# Autodesk Inventor assembly: ASY PNS 1780 FDS 1200x90 Top elbow
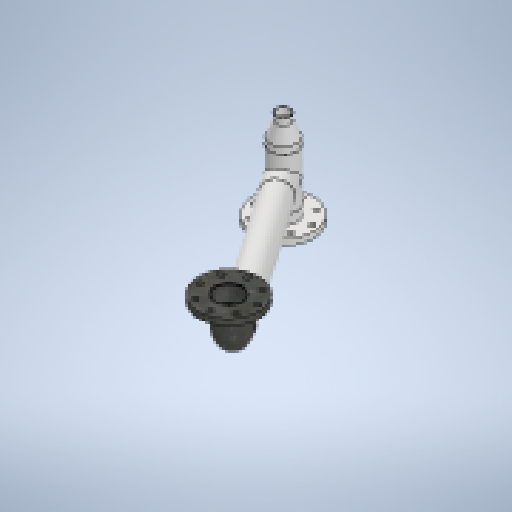
[picture p0: Inventor's stored thumbnail of the model, 512x512]
Saved by Autodesk Inventor 2025.1 (Build 291241020, 241B)
## iProperties
Created: 2025-07-10
Part Number: ASY PNS 1780 FDS 1200x90 Top elbow
Document SubType Name: Assembly
Designer: user
Author: user
## Documents named in this file (7)
- C:\Users\user\YandexDisk-badmisterfox\home pc\Inventor\PNS2-Panaevsk\Filter D1200\ASY PNS 1780 FDS 1200x90 Top elbow.iam
- C:\Users\user\YandexDisk-badmisterfox\home pc\Inventor\PNS2-Panaevsk\Filter D1000\DIN 2576 Slip-On Flange for Welding Series 1 (ISO) - PN 10 80 x 88.9.ipt
- C:\Users\user\YandexDisk-badmisterfox\home pc\Inventor\PNS2-Panaevsk\CC\en-US\DIN 2615-1 T\DIN 2615-1 Tee 88.9 x 5.6 S.ipt
- C:\Users\user\YandexDisk-badmisterfox\home pc\Inventor\PNS2-Panaevsk\Filter D1200\PNS 1722 FDS  tube 1.ipt
- C:\Users\user\YandexDisk-badmisterfox\home pc\Inventor\PNS2-Panaevsk\CC\en-US\DIN 2616 CR (K)\DIN 2616 Concentric Reducer (K) 88.9 x 2.3 - 48.3 x 2.ipt
- C:\Users\user\YandexDisk-badmisterfox\home pc\Inventor\PNS2-Panaevsk\Filter D1200\PNS 1705 FDS tube 1.ipt
- C:\Users\user\YandexDisk-badmisterfox\home pc\Inventor\PNS2-Panaevsk\CC\en-US\JIS B 2312 90 (2)\JIS B 2312 90 Deg Long Elbow Steel 80A x Sch 40.ipt
## Components (8 placed, 6 different names)
1. DIN 2576 Slip-On Flange for Welding Series 1 (ISO) - PN 10 80 x 88.9.ipt:1
2. DIN 2615-1 Tee 88.9 x 5.6 S.ipt:1
3. PNS 1722 FDS  tube 1.ipt:1
4. DIN 2616 Concentric Reducer (K) 88.9 x 2.3 - 48.3 x 2.ipt:1
5. PNS 753 FDS tube.ipt:1
6. JIS B 2312 90 Deg Long Elbow Steel 80A x Sch 40.ipt:1
7. PNS 1722 FDS  tube 1.ipt:2
8. DIN 2576 Slip-On Flange for Welding Series 1 (ISO) - PN 10 80 x 88.9.ipt:2
## Relationships (7: WeldJoint 6, RevoluteJoint 1)
- [RevoluteJoint]: DIN 2615-1 Tee 88.9 x 5.6 S.ipt:1 ↔ PNS 1722 FDS  tube 1.ipt:1
- [WeldJoint]: DIN 2576 Slip-On Flange for Welding Series 1 (ISO) - PN 10 80 x 88.9.ipt:1 ↔ PNS 1722 FDS  tube 1.ipt:1
- [WeldJoint]: DIN 2615-1 Tee 88.9 x 5.6 S.ipt:1 ↔ DIN 2616 Concentric Reducer (K) 88.9 x 2.3 - 48.3 x 2.ipt:1
- [WeldJoint]: DIN 2615-1 Tee 88.9 x 5.6 S.ipt:1 ↔ PNS 753 FDS tube.ipt:1
- [WeldJoint]: PNS 753 FDS tube.ipt:1 ↔ JIS B 2312 90 Deg Long Elbow Steel 80A x Sch 40.ipt:1
- [WeldJoint]: JIS B 2312 90 Deg Long Elbow Steel 80A x Sch 40.ipt:1 ↔ PNS 1722 FDS  tube 1.ipt:2
- [WeldJoint]: PNS 1722 FDS  tube 1.ipt:2 ↔ DIN 2576 Slip-On Flange for Welding Series 1 (ISO) - PN 10 80 x 88.9.ipt:2
## Named parameters: d74_d69 = 0 mm, d75_d70 = 180 deg, d76_d71 = 0 mm, d77_d72 = 0 mm
